# Autodesk Inventor assembly: OBG-Dribbler
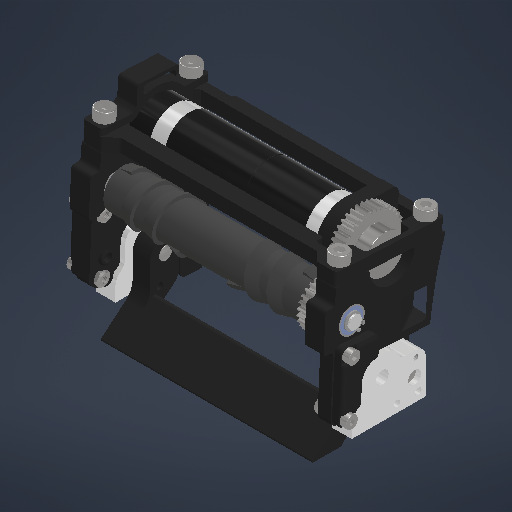
[picture p0: Inventor's stored thumbnail of the model, 512x512]
Saved by Autodesk Inventor 2025.2 (Build 292293000, 293)
## iProperties
Created: 2024-11-26
Part Number: OBG-Dribbler
Document SubType Name: Assembly
Designer: Fabian
Mass: 66.035 g
Surface Area: 342.991 cm^2
Volume: 48.8958 cm^3
Density: 1.35053 g/cm^3
Author: Fabian
## Documents named in this file (24)
- C:\Users\Faabs\Desktop\HBG v2025\Oberbaugruppen\OBG-Dribbler\OBG-Dribbler.iam
- C:\Users\Faabs\Desktop\HBG v2025\Oberbaugruppen\OBG-Dribbler\Bauteile\Lagerblock.ipt
- C:\Users\Faabs\Desktop\HBG v2025\Oberbaugruppen\OBG-Dribbler\Bauteile\Seitenplatte.ipt
- C:\Users\Faabs\Desktop\HBG v2025\Oberbaugruppen\OBG-Dribbler\Bauteile\Seitenplatte_MIR.ipt
- C:\Users\Faabs\Desktop\HBG v2025\Oberbaugruppen\OBG-Dribbler\Bauteile\Schaufel.ipt
- C:\Users\Faabs\Desktop\HBG v2025\Verbindungselemente\ISO 8745\ISO 8745 - 4 x 10.ipt
- C:\Users\Faabs\Desktop\HBG v2025\Oberbaugruppen\OBG-Dribbler\Bauteile\38z.ipt
- C:\Users\Faabs\Desktop\HBG v2025\Oberbaugruppen\OBG-Dribbler\Bauteile\26z.ipt
- C:\Users\Faabs\Desktop\HBG v2025\Oberbaugruppen\OBG-Dribbler\Bauteile\Maxon EC-16 30W\Maxon EC-16 30W.iam
- C:\Users\Faabs\Desktop\HBG v2025\Oberbaugruppen\OBG-Dribbler\Bauteile\Motorhalterung.ipt
- C:\Users\Faabs\Desktop\HBG v2025\Verbindungselemente\DIN 912\DIN 912 - M3 x 0,5 x 10 x 8,75.ipt
- C:\Users\Faabs\Desktop\HBG v2025\Oberbaugruppen\OBG-Dribbler\Bauteile\Welle.ipt
- C:\Users\Faabs\Desktop\HBG v2025\Oberbaugruppen\OBG-Dribbler\Bauteile\Kugellager 8 x 4 x 3.ipt
- C:\Users\Faabs\Desktop\HBG v2025\Verbindungselemente\DIN 471\DIN 471-SR-FST\DIN 471-SR-FST\DIN 471-SR-FST.ipt
- C:\Users\Faabs\Desktop\HBG v2025\Oberbaugruppen\OBG-Dribbler\Bauteile\Rahmen.ipt
- C:\Users\Faabs\Desktop\HBG v2025\Verbindungselemente\DIN 912\DIN 912 - M3 x 0,5 x 6 x 4,75.ipt
- C:\Users\Faabs\Desktop\HBG v2025\Oberbaugruppen\OBG-Dribbler\Bauteile\Kabelklemme.ipt
- C:\Users\Faabs\Desktop\HBG v2025\Oberbaugruppen\OBG-Dribbler\Bauteile\Schnecke.ipt
- C:\Users\Faabs\Desktop\HBG v2025\Verbindungselemente\ISO 14581\ISO 14581 - M2x5-8.8.ipt
- C:\Users\Faabs\Desktop\HBG v2025\Platinen\Lichtschranke\Lichtschrankenplatine.ipt
- C:\Users\Faabs\Desktop\HBG v2025\Oberbaugruppen\OBG-Dribbler\Bauteile\LS-Abdeckung.ipt
- C:\Users\Faabs\Desktop\HBG v2025\Verbindungselemente\DIN 912\DIN 912 - M2 x 0,4 x 6 x 5.ipt
- C:\Users\Faabs\Desktop\HBG v2025\Oberbaugruppen\OBG-Dribbler\Bauteile\LS-Abdeckung_MIR.ipt
- C:\Users\Faabs\Desktop\HBG v2025\Verbindungselemente\ISO 4032\ISO 4032 - M2 - ISO.ipt
## Components (47 placed, 23 different names)
1. Schnecke:1 — Passend:72, Passend:73
2. 26z:1 — Fluchtend:4, Passend:36, Passend:73
3. Welle:1 — Passend:39, Fluchtend:5, Passend:47, Passend:48, Passend:49, Passend:50, Passend:72
4. DIN 471-SR-FST:1 — Passend:47, Passend:48
5. DIN 471-SR-FST:2 — Passend:49, Passend:50
6. Kugellager 8 x 4 x 3:1 — Passend:43, Fluchtend:7
7. Kugellager 8 x 4 x 3:2 — Passend:44, Fluchtend:6
8. Kugellager 8 x 4 x 3:3 — Passend:45, Fluchtend:8
9. Kugellager 8 x 4 x 3:4 — Passend:46, Fluchtend:9
10. Chip Schaufel v2:1 — Passend:12, Einfügen:5, Einfügen:6, Winkel:2, Passend:103
11. Rahmen:1 — Passend:57, Passend:60, Passend:61, Passend:64, Passend:65, Passend:66, Passend:71, Einfügen:40, Einfügen:41
12. Lagerblock:2 — Fluchtend:1, Passend:1, Passend:2, Passend:8, Passend:17
13. Lagerblock:3 — Fluchtend:1, Passend:1, Passend:2, Passend:3, Fluchtend:2, Passend:4, Passend:7, Passend:12, Passend:16, Winkel:1, Passend:70, Winkel:2, Passend:103
14. Seitenplatte:1 — Passend:7, Fluchtend:3, Passend:36, Passend:39, Fluchtend:5, Passend:43, Passend:44, Fluchtend:6, Fluchtend:7, Winkel:1, Passend:54, Passend:60, Passend:62, Passend:63, Passend:71, Passend:93, Passend:94, Passend:95, Passend:99, Passend:106, Passend:107, Passend:108, Passend:109, Passend:114, Passend:115
15. Seitenplatte_MIR:1 — Passend:8, Fluchtend:3, Passend:45, Passend:46, Fluchtend:8, Fluchtend:9, Passend:57, Passend:61, Passend:96, Passend:97, Passend:98, Passend:104, Passend:105, Passend:110, Passend:111, Passend:112, Passend:113
16. Kabelklemme:1 — Passend:64, Passend:65, Passend:66, Einfügen:28, Einfügen:29
17. Maxon EC-16 30W:1 [sub-assembly] — Passend:35, Passend:90, Passend:92
18. Motorhalterung:1 — Passend:32, Passend:54, Passend:62, Passend:63, Passend:90, Einfügen:32, Einfügen:33, Passend:92, Einfügen:42, Einfügen:43, Einfügen:44, Einfügen:45, Einfügen:46, Einfügen:47
19. 38z:1 — Passend:32, Passend:35, Fluchtend:4
20. Lichtschrankenplatine:1 — Passend:93, Passend:94, Passend:95, Passend:100, Passend:101, Passend:102
21. Lichtschrankenplatine:2 — Passend:96, Passend:97, Passend:98
22. LS-Abdeckung:1 — Passend:100, Passend:101, Passend:102, Einfügen:48, Einfügen:49
23. LS-Abdeckung_MIR:1 — Einfügen:50, Einfügen:51
24. DIN 912 - ersetzt durch DIN EN ISO 4762 M2 x 6:1 — Einfügen:48
25. DIN 912 - ersetzt durch DIN EN ISO 4762 M2 x 6:2 — Einfügen:49
26. DIN 912 - ersetzt durch DIN EN ISO 4762 M2 x 6:3 — Einfügen:50
27. DIN 912 - ersetzt durch DIN EN ISO 4762 M2 x 6:4 — Einfügen:51
28. DIN 912 - ersetzt durch DIN EN ISO 4762 M3 x 6:4 — Einfügen:40
29. DIN 912 - ersetzt durch DIN EN ISO 4762 M3 x 6:3 — Einfügen:29
30. DIN 912 - ersetzt durch DIN EN ISO 4762 M3 x 6:2 — Einfügen:28
31. DIN 912 - ersetzt durch DIN EN ISO 4762 M3 x 6:1 — Einfügen:41
32. DIN 912 - ersetzt durch DIN EN ISO 4762 M3 x 10:2 — Einfügen:32
33. DIN 912 - ersetzt durch DIN EN ISO 4762 M3 x 10:1 — Einfügen:33
34. ISO 8745 - 4 x 10:4
35. ISO 8745 - 4 x 10:3 — Passend:70, Passend:99
36. ISO 8745 - 4 x 10:2 — Passend:17, Einfügen:5
37. ISO 8745 - 4 x 10:1 — Passend:16, Einfügen:6
38. Schraube ISO 14581:2013(E) M2x5-8.8:1 — Einfügen:47
39. Schraube ISO 14581:2013(E) M2x5-8.8:2 — Einfügen:46
40. Schraube ISO 14581:2013(E) M2x5-8.8:3 — Einfügen:45
41. Schraube ISO 14581:2013(E) M2x5-8.8:4 — Einfügen:42
42. Schraube ISO 14581:2013(E) M2x5-8.8:5 — Einfügen:43
43. Schraube ISO 14581:2013(E) M2x5-8.8:6 — Einfügen:44
44. ISO 4032 M2:4 — Passend:106, Passend:109, Passend:114
45. ISO 4032 M2:3 — Passend:107, Passend:108, Passend:115
46. ISO 4032 M2:2 — Passend:105, Passend:111, Passend:112
47. ISO 4032 M2:1 — Passend:104, Passend:110, Passend:113
## Relationships (88: Mate 59, Insert 18, Flush 9, Angle 2)
- Fluchtend:1 [Flush]: Lagerblock:2 ↔ Lagerblock:3
- Passend:1 [Mate]: Lagerblock:2 ↔ Lagerblock:3
- Passend:2 [Mate] (67.5 mm): Lagerblock:2 ↔ Lagerblock:3
- Passend:3 [Mate]: Lagerblock:3
- Fluchtend:2 [Flush]: Lagerblock:3
- Passend:4 [Mate] (33.75 mm): Lagerblock:3
- Passend:7 [Mate] (0.2 mm): Lagerblock:3 ↔ Seitenplatte:1
- Passend:8 [Mate] (0.2 mm): Lagerblock:2 ↔ Seitenplatte_MIR:1
- Fluchtend:3 [Flush]: Seitenplatte:1 ↔ Seitenplatte_MIR:1
- Passend:12 [Mate]: Chip Schaufel v2:1 ↔ Lagerblock:3
- Passend:16 [Mate]: Lagerblock:3 ↔ ISO 8745 - 4 x 10:1
- Passend:17 [Mate]: Lagerblock:2 ↔ ISO 8745 - 4 x 10:2
- Einfügen:5 [Insert]: Chip Schaufel v2:1 ↔ ISO 8745 - 4 x 10:2
- Einfügen:6 [Insert]: Chip Schaufel v2:1 ↔ ISO 8745 - 4 x 10:1
- Passend:32 [Mate] (0.25 mm): Motorhalterung:1 ↔ 38z:1
- Passend:35 [Mate]: Maxon EC-16 30W:1 ↔ 38z:1
- Fluchtend:4 [Flush]: 26z:1 ↔ 38z:1
- Passend:36 [Mate]: 26z:1 ↔ Seitenplatte:1
- Passend:39 [Mate]: Welle:1 ↔ Seitenplatte:1
- Fluchtend:5 [Flush] (-1.1 mm): Welle:1 ↔ Seitenplatte:1
- Passend:43 [Mate]: Kugellager 8 x 4 x 3:1 ↔ Seitenplatte:1
- Passend:44 [Mate]: Kugellager 8 x 4 x 3:2 ↔ Seitenplatte:1
- Fluchtend:6 [Flush]: Kugellager 8 x 4 x 3:2 ↔ Seitenplatte:1
- Fluchtend:7 [Flush]: Kugellager 8 x 4 x 3:1 ↔ Seitenplatte:1
- Passend:45 [Mate]: Kugellager 8 x 4 x 3:3 ↔ Seitenplatte_MIR:1
- Passend:46 [Mate]: Kugellager 8 x 4 x 3:4 ↔ Seitenplatte_MIR:1
- Fluchtend:8 [Flush]: Kugellager 8 x 4 x 3:3 ↔ Seitenplatte_MIR:1
- Fluchtend:9 [Flush]: Kugellager 8 x 4 x 3:4 ↔ Seitenplatte_MIR:1
- Passend:47 [Mate]: Welle:1 ↔ DIN 471-SR-FST:1
- Passend:48 [Mate] (0.05 mm): Welle:1 ↔ DIN 471-SR-FST:1
- Passend:49 [Mate]: Welle:1 ↔ DIN 471-SR-FST:2
- Passend:50 [Mate] (0.05 mm): Welle:1 ↔ DIN 471-SR-FST:2
- Winkel:1 [Angle] (357.29 deg): Lagerblock:3 ↔ Seitenplatte:1
- Passend:54 [Mate]: Seitenplatte:1 ↔ Motorhalterung:1
- Passend:57 [Mate]: Rahmen:1 ↔ Seitenplatte_MIR:1
- Passend:60 [Mate]: Rahmen:1 ↔ Seitenplatte:1
- Passend:61 [Mate]: Rahmen:1 ↔ Seitenplatte_MIR:1
- Passend:62 [Mate]: Seitenplatte:1 ↔ Motorhalterung:1
- Passend:63 [Mate]: Seitenplatte:1 ↔ Motorhalterung:1
- Passend:64 [Mate]: Rahmen:1 ↔ Kabelklemme:1
- Passend:65 [Mate]: Rahmen:1 ↔ Kabelklemme:1
- Passend:66 [Mate]: Rahmen:1 ↔ Kabelklemme:1
- Einfügen:28 [Insert]: Kabelklemme:1 ↔ DIN 912 - ersetzt durch DIN EN ISO 4762 M3 x 6:2
- Einfügen:29 [Insert]: Kabelklemme:1 ↔ DIN 912 - ersetzt durch DIN EN ISO 4762 M3 x 6:3
- Passend:70 [Mate]: Lagerblock:3 ↔ ISO 8745 - 4 x 10:3
- Passend:71 [Mate]: Rahmen:1 ↔ Seitenplatte:1
- Passend:72 [Mate]: Schnecke:1 ↔ Welle:1
- Passend:73 [Mate]: Schnecke:1 ↔ 26z:1
- Passend:90 [Mate]: Maxon EC-16 30W:1 ↔ Motorhalterung:1
- Einfügen:32 [Insert]: Motorhalterung:1 ↔ DIN 912 - ersetzt durch DIN EN ISO 4762 M3 x 10:2
- Einfügen:33 [Insert]: Motorhalterung:1 ↔ DIN 912 - ersetzt durch DIN EN ISO 4762 M3 x 10:1
- Passend:92 [Mate]: Maxon EC-16 30W:1 ↔ Motorhalterung:1
- Einfügen:40 [Insert]: Rahmen:1 ↔ DIN 912 - ersetzt durch DIN EN ISO 4762 M3 x 6:4
- Einfügen:41 [Insert]: Rahmen:1 ↔ DIN 912 - ersetzt durch DIN EN ISO 4762 M3 x 6:1
- Einfügen:42 [Insert]: Motorhalterung:1 ↔ Schraube ISO 14581:2013(E) M2x5-8.8:4
- Einfügen:43 [Insert]: Motorhalterung:1 ↔ Schraube ISO 14581:2013(E) M2x5-8.8:5
- Einfügen:44 [Insert]: Motorhalterung:1 ↔ Schraube ISO 14581:2013(E) M2x5-8.8:6
- Einfügen:45 [Insert]: Motorhalterung:1 ↔ Schraube ISO 14581:2013(E) M2x5-8.8:3
- Einfügen:46 [Insert]: Motorhalterung:1 ↔ Schraube ISO 14581:2013(E) M2x5-8.8:2
- Einfügen:47 [Insert]: Motorhalterung:1 ↔ Schraube ISO 14581:2013(E) M2x5-8.8:1
- Passend:93 [Mate]: Seitenplatte:1 ↔ Lichtschrankenplatine:1
- Passend:94 [Mate]: Seitenplatte:1 ↔ Lichtschrankenplatine:1
- Passend:95 [Mate]: Seitenplatte:1 ↔ Lichtschrankenplatine:1
- Passend:96 [Mate]: Seitenplatte_MIR:1 ↔ Lichtschrankenplatine:2
- Passend:97 [Mate]: Seitenplatte_MIR:1 ↔ Lichtschrankenplatine:2
- Passend:98 [Mate]: Seitenplatte_MIR:1 ↔ Lichtschrankenplatine:2
- Passend:99 [Mate]: Seitenplatte:1 ↔ ISO 8745 - 4 x 10:3
- Passend:100 [Mate]: Lichtschrankenplatine:1 ↔ LS-Abdeckung:1
- Passend:101 [Mate]: Lichtschrankenplatine:1 ↔ LS-Abdeckung:1
- Passend:102 [Mate]: Lichtschrankenplatine:1 ↔ LS-Abdeckung:1
- Einfügen:48 [Insert]: LS-Abdeckung:1 ↔ DIN 912 - ersetzt durch DIN EN ISO 4762 M2 x 6:1
- Einfügen:49 [Insert]: LS-Abdeckung:1 ↔ DIN 912 - ersetzt durch DIN EN ISO 4762 M2 x 6:2
- Winkel:2 [Angle] (0 deg): Chip Schaufel v2:1 ↔ Lagerblock:3
- Passend:103 [Mate] (0.85 mm): Chip Schaufel v2:1 ↔ Lagerblock:3
- Einfügen:50 [Insert]: LS-Abdeckung_MIR:1 ↔ DIN 912 - ersetzt durch DIN EN ISO 4762 M2 x 6:3
- Einfügen:51 [Insert]: LS-Abdeckung_MIR:1 ↔ DIN 912 - ersetzt durch DIN EN ISO 4762 M2 x 6:4
- Passend:104 [Mate]: Seitenplatte_MIR:1 ↔ ISO 4032 M2:1
- Passend:105 [Mate]: Seitenplatte_MIR:1 ↔ ISO 4032 M2:2
- Passend:106 [Mate]: Seitenplatte:1 ↔ ISO 4032 M2:4
- Passend:107 [Mate]: Seitenplatte:1 ↔ ISO 4032 M2:3
- Passend:108 [Mate]: Seitenplatte:1 ↔ ISO 4032 M2:3
- Passend:109 [Mate]: Seitenplatte:1 ↔ ISO 4032 M2:4
- Passend:110 [Mate]: Seitenplatte_MIR:1 ↔ ISO 4032 M2:1
- Passend:111 [Mate]: Seitenplatte_MIR:1 ↔ ISO 4032 M2:2
- Passend:112 [Mate]: Seitenplatte_MIR:1 ↔ ISO 4032 M2:2
- Passend:113 [Mate]: Seitenplatte_MIR:1 ↔ ISO 4032 M2:1
- Passend:114 [Mate]: Seitenplatte:1 ↔ ISO 4032 M2:4
- Passend:115 [Mate]: Seitenplatte:1 ↔ ISO 4032 M2:3
